# Autodesk Inventor assembly: Z
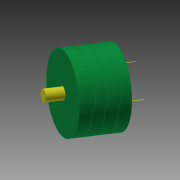
[picture p0: Inventor's stored thumbnail of the model, 180x180]
Saved by Autodesk Inventor 2014 (Build 180170000, 170)
## iProperties
Created: 2013-05-24
Part Number: Z
Document SubType Name: Assembly
Designer: hartmann
Author: hartmann
## Documents named in this file (8)
- C:\Users\Felix\Desktop\Beep\Hardware\Z132053\Z.iam
- C:\Users\Felix\Desktop\Beep\Hardware\Z132053\Z20.ipt
- C:\Users\Felix\Desktop\Beep\Hardware\Z132053\Z13.ipt
- C:\Users\Felix\Desktop\Beep\Hardware\Z132053\PHolderEnd.iam
- C:\Users\Felix\Desktop\Beep\Hardware\Z132053\I53D.ipt
- C:\Users\Felix\Desktop\Beep\Hardware\Z132053\inD.ipt
- C:\Users\Felix\Desktop\EndA.ipt
- C:\Users\Felix\Desktop\PHolderP.ipt
## Components (17 placed, 7 different names)
1. PHolderP:1 — Flush:50, Mate:50, Mate:51, Mate:52, Mate:53, Mate:54, Mate:55, Mate:56
2. Z20:1 — Mate:51, Mate:54
3. Z20:2 — Mate:52, Mate:56
4. Z20:3 — Mate:53, Mate:55
5. PHolderP:2 — Mate:57, Mate:58, Mate:59, Mate:60, Mate:61, Mate:62, Mate:63, Flush:51
6. Z20:4 — Mate:58, Mate:61
7. Z20:5 — Mate:59, Mate:63
8. Z20:6 — Mate:60, Mate:62
9. Z13:1 — Mate:11, Mate:43
10. PHolderEnd:1 [sub-assembly] — Mate:14, Mate:15, Mate:16, Mate:17, Mate:34, Mate:35, Mate:36, Mate:45
11. Z20:7 — Mate:15, Mate:35
12. Z20:8 — Mate:16, Mate:36
13. Z20:9 — Mate:17, Mate:34
14. I53D:1 — Mate:29, Mate:46, Mate:47, Flush:50
15. I53D:2 — Mate:30, Mate:47, Mate:48, Flush:51
16. inD:1 — Mate:31, Mate:43, Mate:48
17. EndA:1 — Mate:44, Mate:45, Mate:46
## Relationships (33: Mate 31, Flush 2)
- Mate:11: Z13:1
- Mate:14: PHolderEnd:1
- Mate:15: PHolderEnd:1 ↔ Z20:7
- Mate:16: PHolderEnd:1 ↔ Z20:8
- Mate:17: PHolderEnd:1 ↔ Z20:9
- Mate:29: I53D:1
- Mate:30: I53D:2
- Mate:31: inD:1
- Mate:34: PHolderEnd:1 ↔ Z20:9
- Mate:35: PHolderEnd:1 ↔ Z20:7
- Mate:36: PHolderEnd:1 ↔ Z20:8
- Mate:43: Z13:1 ↔ inD:1
- Mate:44: EndA:1
- Mate:45: PHolderEnd:1 ↔ EndA:1
- Mate:46: I53D:1 ↔ EndA:1
- Mate:47: I53D:1 ↔ I53D:2
- Mate:48: I53D:2 ↔ inD:1
- Flush:50: PHolderP:1 ↔ I53D:1
- Mate:50: PHolderP:1
- Mate:51: PHolderP:1 ↔ Z20:1
- Mate:52: PHolderP:1 ↔ Z20:2
- Mate:53: PHolderP:1 ↔ Z20:3
- Mate:54: PHolderP:1 ↔ Z20:1
- Mate:55: PHolderP:1 ↔ Z20:3
- Mate:56: PHolderP:1 ↔ Z20:2
- Mate:57: PHolderP:2
- Mate:58: PHolderP:2 ↔ Z20:4
- Mate:59: PHolderP:2 ↔ Z20:5
- Mate:60: PHolderP:2 ↔ Z20:6
- Mate:61: PHolderP:2 ↔ Z20:4
- Mate:62: PHolderP:2 ↔ Z20:6
- Mate:63: PHolderP:2 ↔ Z20:5
- Flush:51: PHolderP:2 ↔ I53D:2
